# Autodesk Inventor assembly: Zespół1
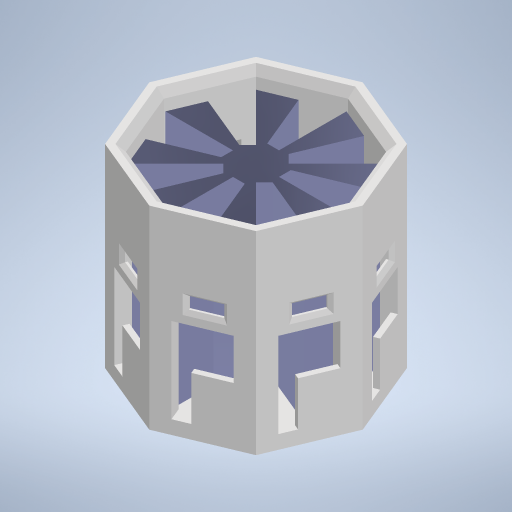
[picture p0: Inventor's stored thumbnail of the model, 512x512]
Saved by Autodesk Inventor 2023 (Build 270158000, 158)
## iProperties
Created: 2022-05-03
Part Number: Zespół1
Document SubType Name: Assembly
Designer: Ciućmok
Author: Ciućmok
## Documents named in this file (3)
- C:\Users\Ciućmok\Desktop\SDUP_obu\Zespół1.iam
- C:\Users\Ciućmok\Desktop\SDUP_obu\body_main.ipt
- C:\Users\Ciućmok\Desktop\SDUP_obu\dopychacz.ipt
## Components (2 placed, 2 different names)
1. body_main:1 — Równoległe:1, Równoległe:2
2. dopychacz:1 — Równoległe:1, Równoległe:2
## Relationships (2: Flush 2)
- Równoległe:1 [Flush]: body_main:1 ↔ dopychacz:1
- Równoległe:2 [Flush]: body_main:1 ↔ dopychacz:1
